# Autodesk Inventor assembly: Rod下
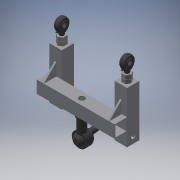
[picture p0: Inventor's stored thumbnail of the model, 180x180]
Saved by Autodesk Inventor 2018 (Build 220112000, 112)
## iProperties
Created: 2017-09-13
Part Number: Rod下
Material: 一般
Document SubType Name: Assembly
Designer: mura5
Author: mura5
## Documents named in this file (8)
- D:\Works\RBBR\CAD\サスペンション\下アーム(前後).iam
- D:\Works\RBBR\CAD\サスペンション\PipeB蓋.ipt
- D:\Works\RBBR\CAD\汎用部品\M12_1種ナット.ipt
- D:\Works\RBBR\CAD\サスペンション\PipeB(前,上).ipt
- D:\Works\RBBR\CAD\サスペンション\リブ.ipt
- D:\Works\RBBR\CAD\サスペンション\アームはり(前).ipt
- D:\Works\RBBR\CAD\汎用部品\ピロボール12mm\POS 12.iam
- D:\Works\RBBR\CAD\汎用部品\エルボール14mm\LHSA 14.iam
## Components (14 placed, 7 different names)
1. PipeB(前,上):1 — リジッド:10, フラッシュ:4, メイト:3, メイト:7, 角度:2
2. PipeB蓋:1 — リジッド:2, リジッド:10, 回転:1, フラッシュ:3
3. M12_1種ナット:1 — リジッド:2, リジッド:3
4. M12_1種ナット:2 — リジッド:3
5. アームはり(前):1 — フラッシュ:1, フラッシュ:3, フラッシュ:4, メイト:3, メイト:4, フラッシュ:5, メイト:6, フラッシュ:6, メイト:8, フラッシュ:7, リジッド:11
6. PipeB(前,上):2 — リジッド:9, メイト:4, フラッシュ:5, メイト:5, 角度:1
7. PipeB蓋:2 — リジッド:7, リジッド:9, 回転:2, フラッシュ:1
8. M12_1種ナット:3 — リジッド:7, リジッド:8
9. M12_1種ナット:4 — リジッド:8
10. リブ:1 — メイト:5, メイト:6, フラッシュ:6
11. リブ:2 — メイト:7, メイト:8, フラッシュ:7
12. POS 12:1 [sub-assembly] — 回転:1, 角度:2
13. POS 12:2 [sub-assembly] — 回転:2, 角度:1
14. LHSA 14:1 [sub-assembly] — リジッド:11
## Relationships (23: WeldJoint 7, Flush 6, Mate 6, RevoluteJoint 2, Angle 2)
- リジッド:2 [WeldJoint]: PipeB蓋:1 ↔ M12_1種ナット:1
- リジッド:3 [WeldJoint]: M12_1種ナット:1 ↔ M12_1種ナット:2
- リジッド:7 [WeldJoint]: PipeB蓋:2 ↔ M12_1種ナット:3
- リジッド:8 [WeldJoint]: M12_1種ナット:3 ↔ M12_1種ナット:4
- リジッド:9 [WeldJoint]: PipeB(前,上):2 ↔ PipeB蓋:2
- リジッド:10 [WeldJoint]: PipeB(前,上):1 ↔ PipeB蓋:1
- フラッシュ:1 [Flush] (65 mm): アームはり(前):1 ↔ PipeB蓋:2
- フラッシュ:3 [Flush] (65 mm): PipeB蓋:1 ↔ アームはり(前):1
- フラッシュ:4 [Flush]: PipeB(前,上):1 ↔ アームはり(前):1
- メイト:3 [Mate]: PipeB(前,上):1 ↔ アームはり(前):1
- メイト:4 [Mate]: アームはり(前):1 ↔ PipeB(前,上):2
- フラッシュ:5 [Flush]: アームはり(前):1 ↔ PipeB(前,上):2
- メイト:5 [Mate]: PipeB(前,上):2 ↔ リブ:1
- メイト:6 [Mate]: アームはり(前):1 ↔ リブ:1
- フラッシュ:6 [Flush] (13.75 mm): アームはり(前):1 ↔ リブ:1
- メイト:7 [Mate]: PipeB(前,上):1 ↔ リブ:2
- メイト:8 [Mate]: アームはり(前):1 ↔ リブ:2
- フラッシュ:7 [Flush] (13.75 mm): アームはり(前):1 ↔ リブ:2
- 回転:1 [RevoluteJoint] (10 mm): PipeB蓋:1 ↔ POS 12:1
- 回転:2 [RevoluteJoint] (10 mm): PipeB蓋:2 ↔ POS 12:2
- 角度:1 [Angle] (0 deg): PipeB(前,上):2 ↔ POS 12:2
- 角度:2 [Angle] (0 deg): PipeB(前,上):1 ↔ POS 12:1
- リジッド:11 [WeldJoint]: アームはり(前):1 ↔ LHSA 14:1
